# Autodesk Inventor assembly: Złożenie platformy
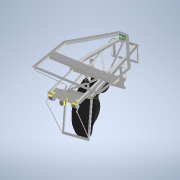
[picture p0: Inventor's stored thumbnail of the model, 180x180]
Saved by Autodesk Inventor 2021 (Build 250183000, 183)
## iProperties
Created: 2022-04-07
Part Number: Złożenie platformy
Document SubType Name: Assembly
Designer: Łukasz
d107: -146,04 deg
d55: -41,15 deg
d53: -130,37 deg
Author: Łukasz
## Documents named in this file (15)
- E:\Pliki inventor i stl\motion platform\Złożenie platformy.iam
- E:\Pliki inventor i stl\motion platform\rama pod fotel.ipt
- E:\Pliki inventor i stl\motion platform\seat.ipt
- E:\Pliki inventor i stl\motion platform\Universal joint\universal joint assembly.iam
- E:\Pliki inventor i stl\motion platform\rama pośrednia.ipt
- E:\Pliki inventor i stl\motion platform\20mm_P_bearing.ipt
- E:\Pliki inventor i stl\motion platform\rama podstawa.ipt
- E:\Pliki inventor i stl\motion platform\CNS 8279 - 20 - 100.ipt
- E:\Pliki inventor i stl\motion platform\silnik 1016\Moteur DC - MY1016.iam
- E:\Pliki inventor i stl\motion platform\cięgno silnika platformy.ipt
- E:\Pliki inventor i stl\motion platform\przegub 8mm\RJ-8-501.iam
- E:\Pliki inventor i stl\motion platform\cięgno fotela.ipt
- E:\Pliki inventor i stl\motion platform\cięgno traction loss.ipt
- E:\Pliki inventor i stl\motion platform\ramie cięgna traction loss.ipt
- E:\Pliki inventor i stl\motion platform\kólko od deskorolki.ipt
## Components (27 placed, 14 different names)
1. rama pod fotel:1 — Rotational:1, Mate:1, Flush:1, Flush:2, Angle:4, Angle:5, Rotational:13, Rotational:14
2. seat:1 — Mate:1, Flush:1, Flush:2
3. universal joint assembly:1 [sub-assembly] — Rotational:1, Angle:2, Mate:3, Insert:1, Angle:5
4. rama pośrednia:1 — Angle:2, Rotational:3, Rotational:4, Mate:2, Angle:4, Mate:3, Insert:1, Rotational:9, Mate:4, Rotational:10, Mate:5, Rotational:23, Angle:6, Flush:4, Rotational:26, Rotational:27, Rotational:28, Rotational:29
5. 20mm_P_bearing:1 — Rotational:3, Rotational:4, Cylindrical:1
6. rama podstawa:1 — Rotational:6, Rotational:7, Mate:2, Rotational:20
7. 20mm_P_bearing:2 — Rotational:6, Rotational:7, Rotational:8
8. CNS 8279 - 20 - 100:1 — Rotational:8, Cylindrical:1
9. Moteur DC - MY1016:1 [sub-assembly] — Rotational:10, Mate:5, Rotational:12
10. Moteur DC - MY1016:2 [sub-assembly] — Rotational:9, Mate:4, Rotational:11
11. cięgno silnika platformy:1 — Rotational:12, Rotational:15
12. cięgno silnika platformy:2 — Rotational:11, Rotational:16
13. RJ-8-501:1 [sub-assembly] — Rotational:13, Rotational:17
14. RJ-8-501:2 [sub-assembly] — Rotational:16, Rotational:18
15. RJ-8-501:3 [sub-assembly] — Rotational:14, Rotational:19
16. RJ-8-501:4 [sub-assembly] — Rotational:15, Rigid:1
17. cięgno fotela:1 — Rotational:18, Rotational:19
18. cięgno fotela:2 — Rigid:1, Rotational:17
19. Moteur DC - MY1016:3 [sub-assembly] — Rotational:23, Angle:6, Flush:3, Rotational:24
20. cięgno traction loss:1 — Rotational:21, Rotational:22
21. RJ-8-501:5 [sub-assembly] — Rotational:20, Rotational:22
22. RJ-8-501:6 [sub-assembly] — Rotational:21, Rotational:25
23. ramie cięgna traction loss:1 — Rotational:24, Rotational:25
24. kólko od deskorolki:1 — Rotational:27
25. kólko od deskorolki:2 — Rotational:28
26. kólko od deskorolki:3 — Rotational:29
27. kólko od deskorolki:4 — Rotational:26
## Relationships (43: RevoluteJoint 27, Mate 5, Flush 4, Angle 4, CylindricalJoint 1, Insert 1, WeldJoint 1)
- Rotational:1 [RevoluteJoint]: rama pod fotel:1 ↔ universal joint assembly:1
- Mate:1 (50 mm): rama pod fotel:1 ↔ seat:1
- Flush:1 (100 mm): rama pod fotel:1 ↔ seat:1
- Flush:2 (115 mm): rama pod fotel:1 ↔ seat:1
- Angle:2 (0 deg): universal joint assembly:1 ↔ rama pośrednia:1
- Rotational:3 [RevoluteJoint]: rama pośrednia:1 ↔ 20mm_P_bearing:1
- Rotational:4 [RevoluteJoint]: rama pośrednia:1 ↔ 20mm_P_bearing:1
- Rotational:6 [RevoluteJoint]: rama podstawa:1 ↔ 20mm_P_bearing:2
- Rotational:7 [RevoluteJoint]: rama podstawa:1 ↔ 20mm_P_bearing:2
- Mate:2 (15 mm): rama pośrednia:1 ↔ rama podstawa:1
- Rotational:8 [RevoluteJoint]: 20mm_P_bearing:2 ↔ CNS 8279 - 20 - 100:1
- Cylindrical:1: 20mm_P_bearing:1 ↔ CNS 8279 - 20 - 100:1
- Angle:4 (0 deg): rama pod fotel:1 ↔ rama pośrednia:1
- Mate:3: universal joint assembly:1 ↔ rama pośrednia:1
- Insert:1: universal joint assembly:1 ↔ rama pośrednia:1
- Angle:5 (0 deg): rama pod fotel:1 ↔ universal joint assembly:1
- Rotational:9 [RevoluteJoint]: rama pośrednia:1 ↔ Moteur DC - MY1016:2
- Mate:4: rama pośrednia:1 ↔ Moteur DC - MY1016:2
- Rotational:10 [RevoluteJoint]: rama pośrednia:1 ↔ Moteur DC - MY1016:1
- Mate:5: rama pośrednia:1 ↔ Moteur DC - MY1016:1
- Rotational:11 [RevoluteJoint]: Moteur DC - MY1016:2 ↔ cięgno silnika platformy:2
- Rotational:12 [RevoluteJoint]: Moteur DC - MY1016:1 ↔ cięgno silnika platformy:1
- Rotational:13 [RevoluteJoint]: rama pod fotel:1 ↔ RJ-8-501:1
- Rotational:14 [RevoluteJoint]: rama pod fotel:1 ↔ RJ-8-501:3
- Rotational:15 [RevoluteJoint]: cięgno silnika platformy:1 ↔ RJ-8-501:4
- Rotational:16 [RevoluteJoint]: cięgno silnika platformy:2 ↔ RJ-8-501:2
- Rigid:1 [WeldJoint]: RJ-8-501:4 ↔ cięgno fotela:2
- Rotational:17 [RevoluteJoint]: RJ-8-501:1 ↔ cięgno fotela:2
- Rotational:18 [RevoluteJoint]: RJ-8-501:2 ↔ cięgno fotela:1
- Rotational:19 [RevoluteJoint]: RJ-8-501:3 ↔ cięgno fotela:1
- Rotational:20 [RevoluteJoint]: rama podstawa:1 ↔ RJ-8-501:5
- Rotational:21 [RevoluteJoint]: cięgno traction loss:1 ↔ RJ-8-501:6
- Rotational:22 [RevoluteJoint]: cięgno traction loss:1 ↔ RJ-8-501:5
- Rotational:23 [RevoluteJoint]: rama pośrednia:1 ↔ Moteur DC - MY1016:3
- Angle:6 (0 deg): rama pośrednia:1 ↔ Moteur DC - MY1016:3
- Flush:3: Moteur DC - MY1016:3
- Flush:4: rama pośrednia:1
- Rotational:24 [RevoluteJoint]: Moteur DC - MY1016:3 ↔ ramie cięgna traction loss:1
- Rotational:25 [RevoluteJoint]: RJ-8-501:6 ↔ ramie cięgna traction loss:1
- Rotational:26 [RevoluteJoint] (1 mm): rama pośrednia:1 ↔ kólko od deskorolki:4
- Rotational:27 [RevoluteJoint] (-1 mm): rama pośrednia:1 ↔ kólko od deskorolki:1
- Rotational:28 [RevoluteJoint] (-1 mm): rama pośrednia:1 ↔ kólko od deskorolki:2
- Rotational:29 [RevoluteJoint] (-1 mm): rama pośrednia:1 ↔ kólko od deskorolki:3
